# Autodesk Inventor assembly: PWTR-0122
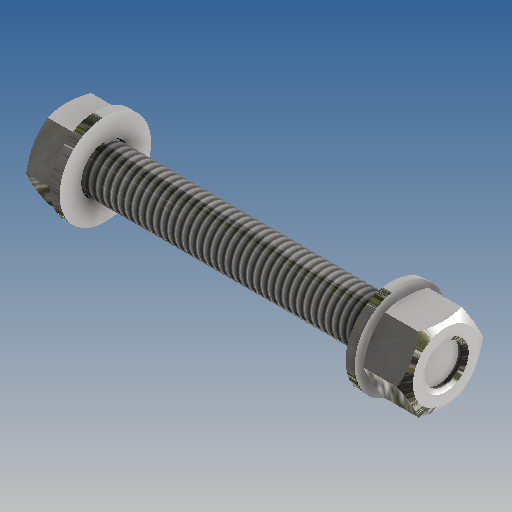
[picture p0: Inventor's stored thumbnail of the model, 512x512]
Saved by Autodesk Inventor 2021.1 (Build 251245000, 245)
## iProperties
Created: 2020-09-02
Part Number: PWTR-0122
Document SubType Name: Assembly
Designer: alid
Description: Arm Fastener
Author: alid
Revision Number: A
## Documents named in this file (4)
- C:\Vault Workspace\Design Data\Projects\PRJ0095\PWTR-Components\PWTR-0122.iam
- C:\Vault Workspace\Design Data\Projects\PRJ0095\PWTR-Components\PWTR-0119.ipt
- C:\Vault Workspace\Design Data\Projects\PRJ0095\PWTR-Components\PWTR-0120.ipt
- C:\Vault Workspace\Design Data\Projects\PRJ0095\PWTR-Components\PWTR-0121.ipt
## Components (4 placed, 3 different names)
1. PWTR-0121:1
2. PWTR-0119:1
3. PWTR-0120:1 — Insert:3
4. PWTR-0120:2 — Insert:3
## Relationships (3: Insert 3)
- [Insert]: PWTR-0121:1 ↔ PWTR-0120:1
- [Insert]: PWTR-0119:1 ↔ PWTR-0120:2
- Insert:3 (50 mm): PWTR-0120:1 ↔ PWTR-0120:2
